# Autodesk Inventor assembly: MarkerHolder
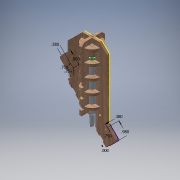
[picture p0: Inventor's stored thumbnail of the model, 180x180]
Saved by Autodesk Inventor 2019 (Build 230136000, 136)
## iProperties
Created: 2019-01-14
Part Number: MarkerHolder
Document SubType Name: Assembly
Designer: nxgam
Author: nxgam
## Documents named in this file (8)
- C:\Users\nxgam\Documents\CAD\Inventor\DiscoDraw\MarkerHolder.iam
- C:\Users\nxgam\Documents\CAD\Inventor\DiscoDraw\MarkerRing.ipt
- C:\Users\nxgam\Documents\CAD\Inventor\DiscoDraw\MarkerShaft.ipt
- C:\Users\nxgam\Documents\CAD\Inventor\DiscoDraw\Imported\expo-marker-1.snapshot.2\EM-COMPLETED MARKER.ipt
- C:\Users\nxgam\Documents\CAD\Inventor\DiscoDraw\MarkerHolderSpacer.ipt
- C:\Users\nxgam\Documents\CAD\Inventor\DiscoDraw\MarkerShaftBottom.ipt
- C:\Users\nxgam\Documents\CAD\Inventor\DiscoDraw\MarkerShaftBot.ipt
- C:\Users\nxgam\Documents\CAD\Inventor\DiscoDraw\MarkerShaftTop2.ipt
## Components (13 placed, 7 different names)
1. MarkerRing:1 — Mate:1, Mate:3, Flush:1, Mate:24, Flush:4, Mate:26
2. MarkerRing:2 — Mate:1, Mate:2, Flush:2, Flush:3, Mate:19, Mate:23, Mate:34
3. MarkerRing:3 — Mate:2, Flush:1, Flush:2, Mate:33
4. MarkerRing:4 — Mate:3, Flush:3, Mate:29, Mate:30, Mate:31, Mate:32, Mate:35, Mate:36, Mate:37
5. MarkerShaft:2 — Flush:5, Mate:29, Flush:6, Mate:30, Mate:33, Flush:8
6. MarkerShaft:3 — Mate:25, Mate:26, Flush:5, Flush:6, Mate:31, Mate:32, Mate:34
7. MarkerShaftBottom:1
8. EM-COMPLETED MARKER:1 — Mate:19
9. MarkerHolderSpacer:1 — Mate:20, Mate:22
10. MarkerHolderSpacer:2 — Mate:20, Mate:22, Mate:23
11. MarkerRing:5 — Mate:24, Flush:4, Mate:25
12. MarkerShaftBot:1 — Flush:7, Flush:8, Mate:35, Flush:9
13. MarkerShaftTop2:1 — Flush:7, Flush:9, Mate:36, Mate:37
## Relationships (28: Mate 19, Flush 9)
- Mate:1: MarkerRing:1 ↔ MarkerRing:2
- Mate:2: MarkerRing:2 ↔ MarkerRing:3
- Mate:3: MarkerRing:1 ↔ MarkerRing:4
- Flush:1: MarkerRing:1 ↔ MarkerRing:3
- Flush:2: MarkerRing:2 ↔ MarkerRing:3
- Flush:3: MarkerRing:2 ↔ MarkerRing:4
- Mate:19: MarkerRing:2 ↔ EM-COMPLETED MARKER:1
- Mate:20: MarkerHolderSpacer:1 ↔ MarkerHolderSpacer:2
- Mate:22: MarkerHolderSpacer:1 ↔ MarkerHolderSpacer:2
- Mate:23: MarkerRing:2 ↔ MarkerHolderSpacer:2
- Mate:24: MarkerRing:1 ↔ MarkerRing:5
- Flush:4: MarkerRing:1 ↔ MarkerRing:5
- Mate:25: MarkerShaft:3 ↔ MarkerRing:5
- Mate:26: MarkerRing:1 ↔ MarkerShaft:3
- Flush:5: MarkerShaft:2 ↔ MarkerShaft:3
- Mate:29: MarkerRing:4 ↔ MarkerShaft:2
- Flush:6: MarkerShaft:2 ↔ MarkerShaft:3
- Mate:30: MarkerRing:4 ↔ MarkerShaft:2
- Mate:31: MarkerRing:4 ↔ MarkerShaft:3
- Mate:32: MarkerRing:4 ↔ MarkerShaft:3
- Mate:33: MarkerRing:3 ↔ MarkerShaft:2
- Mate:34: MarkerRing:2 ↔ MarkerShaft:3
- Flush:7: MarkerShaftBot:1 ↔ MarkerShaftTop2:1
- Flush:8: MarkerShaft:2 ↔ MarkerShaftBot:1
- Mate:35: MarkerRing:4 ↔ MarkerShaftBot:1
- Flush:9: MarkerShaftBot:1 ↔ MarkerShaftTop2:1
- Mate:36: MarkerRing:4 ↔ MarkerShaftTop2:1
- Mate:37: MarkerRing:4 ↔ MarkerShaftTop2:1
